# Autodesk Inventor assembly: assembly_holder3
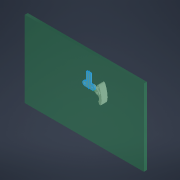
[picture p0: Inventor's stored thumbnail of the model, 180x180]
Saved by Autodesk Inventor 2021 (Build 250183000, 183)
## iProperties
Created: 2021-06-13
Part Number: assembly_holder3
Document SubType Name: Assembly
Designer: Watchdog
Author: Watchdog
## Documents named in this file (5)
- C:\Users\Watchdog\OneDrive - Flinders\Advn Mech Design Shared\6_Development\2_Design\inventor\securing_mechanism\securingMechanism_variant_vertical_x\assembly_holder3.iam
- C:\Users\Watchdog\OneDrive - Flinders\Advn Mech Design Shared\6_Development\2_Design\inventor\securing_mechanism\securingMechanism_variant_vertical_x\holder3_l2.ipt
- C:\Users\Watchdog\OneDrive - Flinders\Advn Mech Design Shared\6_Development\2_Design\inventor\securing_mechanism\securingMechanism_variant_vertical_x\holder3_l3.ipt
- C:\Users\Watchdog\OneDrive - Flinders\Advn Mech Design Shared\6_Development\2_Design\inventor\securing_mechanism\securingMechanism_variant_vertical_x\holder3_l4.ipt
- C:\Users\Watchdog\OneDrive - Flinders\Advn Mech Design Shared\6_Development\2_Design\inventor\securing_mechanism\securingMechanism_variant_vertical_x\holder3_l1.ipt
## Components (4 placed, 4 different names)
1. holder3_l1:1 — Mate:5, Mate:6, Angle:1, Mate:8, Mate:10
2. holder3_l2:1 — Mate:4, Mate:10, Mate:12
3. holder3_l3:1 — Mate:4, Mate:9, Mate:11, Mate:12
4. holder3_l4:1 — Mate:8, Angle:2, Mate:9, Mate:11, Mate:13
## Relationships (11: Mate 9, Angle 2)
- Mate:4: holder3_l2:1 ↔ holder3_l3:1
- Mate:5: holder3_l1:1
- Mate:6: holder3_l1:1
- Angle:1 (0 deg): holder3_l1:1
- Mate:8: holder3_l1:1 ↔ holder3_l4:1
- Angle:2 (0 deg): holder3_l4:1
- Mate:9: holder3_l3:1 ↔ holder3_l4:1
- Mate:10: holder3_l1:1 ↔ holder3_l2:1
- Mate:11: holder3_l3:1 ↔ holder3_l4:1
- Mate:12: holder3_l2:1 ↔ holder3_l3:1
- Mate:13 (-12.133 mm): holder3_l4:1
